# Autodesk Inventor assembly: Pushfit-Adapter
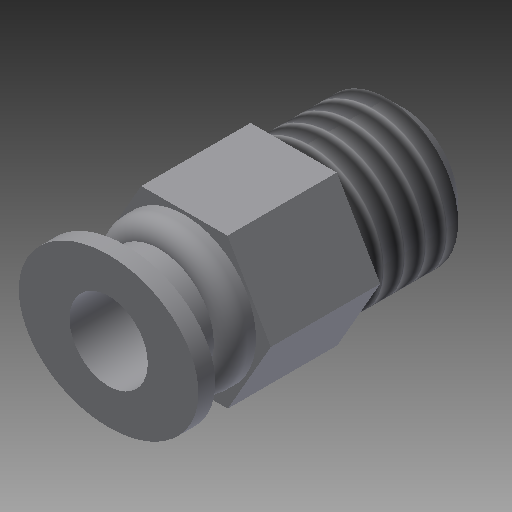
[picture p0: Inventor's stored thumbnail of the model, 512x512]
Saved by Autodesk Inventor 2017 (Build 210142000, 142)
## iProperties
Created: 2016-07-07
Part Number: Pushfit-Adapter
Document SubType Name: Assembly
Designer: joshmamo
Author: joshmamo
## Documents named in this file (3)
- C:\All INVENTOR\SL-Inventor\SL-Beast 3D Printer\Pushfit-Adapter.iam
- C:\All INVENTOR\SL-Inventor\SL-Beast 3D Printer\Pushfit-Adapter.ipt
- C:\All INVENTOR\SL-Inventor\SL-Beast 3D Printer\Pushfit-adapter-cap.ipt
## Components (2 placed, 2 different names)
1. Pushfit-Adapter:1 — Flush:1
2. Pushfit-adapter-cap:1 — Flush:1
## Relationships (1: Flush 1)
- Flush:1: Pushfit-Adapter:1 ↔ Pushfit-adapter-cap:1
